# Autodesk Inventor assembly: 足裏_1_1
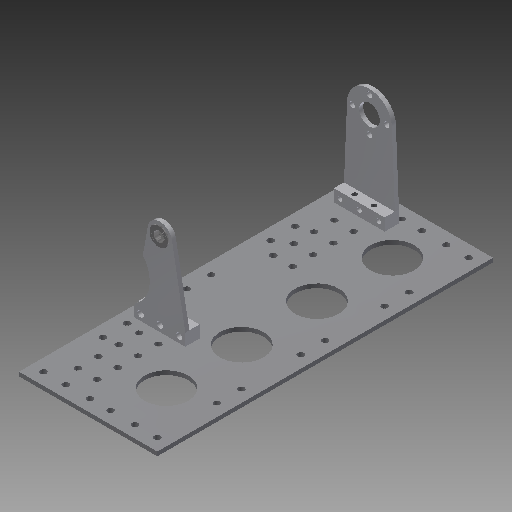
[picture p0: Inventor's stored thumbnail of the model, 512x512]
Saved by Autodesk Inventor 2018 (Build 220112000, 112)
## iProperties
Created: 2016-05-01
Part Number: 足裏_1_1
Document SubType Name: Assembly
Designer: hiroaki
Mass: 45.5975 g
Surface Area: 270.055 cm^2
Volume: 23.2522 cm^3
Density: 1.96099 g/cm^3
Author: hiroaki
## Documents named in this file (6)
- C:\Users\taka\Desktop\OPR\OpenPlatform_ver1_0\下半身\足裏\足裏_1_1.iam
- C:\Users\taka\Desktop\OPR\OpenPlatform_ver1_0\下半身\足裏\足裏_メインフレーム_1_1.ipt
- C:\Users\taka\Desktop\OPR\OpenPlatform_ver1_0\下半身\足裏\足裏_メインフレーム_1_2.ipt
- C:\Users\taka\Desktop\OPR\OpenPlatform_ver1_0\下半身\足裏\足裏_サブフレーム_1_1.ipt
- C:\Users\taka\Desktop\OPR\OpenPlatform_ver1_0\既製品\NSK_RB_MF85ZZ\MF85ZZ.iam
- C:\Users\taka\Desktop\OPR\OpenPlatform_ver1_0\下半身\足裏\足裏_メインフレーム_1_3.ipt
## Components (6 placed, 5 different names)
1. 足裏_メインフレーム_1_1:1 — メイト:1, フラッシュ:1, フラッシュ:2, メイト:2, フラッシュ:3, メイト:3, 挿入:4, 挿入:5, 挿入:6
2. 足裏_メインフレーム_1_2:1 — メイト:2, フラッシュ:3, メイト:3, 挿入:1, 挿入:2, 挿入:3, 挿入:7
3. 足裏_サブフレーム_1_1:1 — 挿入:1, 挿入:2, 挿入:3, 挿入:10, 挿入:11
4. 足裏_サブフレーム_1_1:2 — 挿入:4, 挿入:5, 挿入:6, 挿入:8, 挿入:9
5. MF85ZZ:1 [sub-assembly] — 挿入:7
6. 足裏_メインフレーム_1_3:1 — 挿入:8, 挿入:9, 挿入:10, 挿入:11
## Relationships (17: Insert 11, Mate 3, Flush 3)
- メイト:1 [Mate]: 足裏_メインフレーム_1_1:1
- フラッシュ:1 [Flush]: 足裏_メインフレーム_1_1:1
- フラッシュ:2 [Flush] (50.5 mm): 足裏_メインフレーム_1_1:1
- メイト:2 [Mate]: 足裏_メインフレーム_1_1:1 ↔ 足裏_メインフレーム_1_2:1
- フラッシュ:3 [Flush]: 足裏_メインフレーム_1_1:1 ↔ 足裏_メインフレーム_1_2:1
- メイト:3 [Mate] (101 mm): 足裏_メインフレーム_1_1:1 ↔ 足裏_メインフレーム_1_2:1
- 挿入:1 [Insert]: 足裏_メインフレーム_1_2:1 ↔ 足裏_サブフレーム_1_1:1
- 挿入:2 [Insert]: 足裏_メインフレーム_1_2:1 ↔ 足裏_サブフレーム_1_1:1
- 挿入:3 [Insert]: 足裏_メインフレーム_1_2:1 ↔ 足裏_サブフレーム_1_1:1
- 挿入:4 [Insert]: 足裏_メインフレーム_1_1:1 ↔ 足裏_サブフレーム_1_1:2
- 挿入:5 [Insert]: 足裏_メインフレーム_1_1:1 ↔ 足裏_サブフレーム_1_1:2
- 挿入:6 [Insert]: 足裏_メインフレーム_1_1:1 ↔ 足裏_サブフレーム_1_1:2
- 挿入:7 [Insert]: 足裏_メインフレーム_1_2:1 ↔ MF85ZZ:1
- 挿入:8 [Insert]: 足裏_サブフレーム_1_1:2 ↔ 足裏_メインフレーム_1_3:1
- 挿入:9 [Insert]: 足裏_サブフレーム_1_1:2 ↔ 足裏_メインフレーム_1_3:1
- 挿入:10 [Insert]: 足裏_サブフレーム_1_1:1 ↔ 足裏_メインフレーム_1_3:1
- 挿入:11 [Insert]: 足裏_サブフレーム_1_1:1 ↔ 足裏_メインフレーム_1_3:1
